# Autodesk Inventor assembly: MultiPassSCAN_outsideIn-DFMOD_SCAN_COLOR
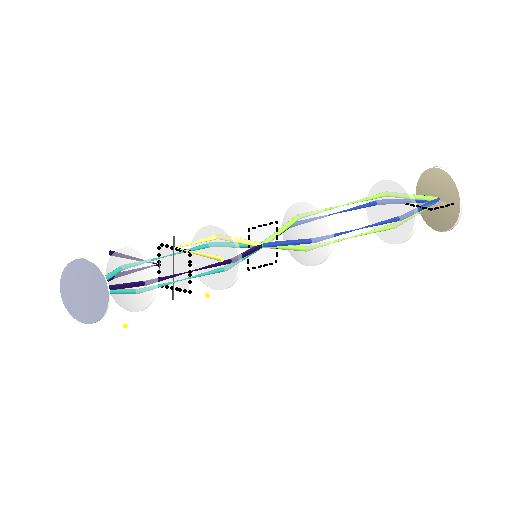
[picture p0: Inventor's stored thumbnail of the model, 512x512]
Saved by Autodesk Inventor 2026.1 (Build 301233000, 233)
## iProperties
Created: 2024-08-19
Part Number: MultiPassSCAN_outsideIn-DFMOD_SCAN_COLOR
Document SubType Name: Assembly
Designer: User
Author: User
## Documents named in this file (22)
- C:\Users\farin012\Downloads\fig4\fig4\MultiPassSCAN_outsideIn-DFMOD_SCAN_COLOR.iam
- C:\Users\farin012\Downloads\fig4\fig4\BB1-E02-Solidworks.ipt
- C:\Users\farin012\Downloads\fig4\fig4\LoopPlane1.ipt
- C:\Users\farin012\Downloads\fig4\fig4\LA1608-AB-Solidworks\LA1608-AB-2LOOP_grid.ipt
- C:\Users\farin012\Downloads\fig4\fig4\LOOP1_COLL.ipt
- C:\Users\farin012\Downloads\fig4\fig4\LOOP1_COLL_PREDEF1.ipt
- C:\Users\farin012\Downloads\fig4\fig4\LOOP1_COLL_POSTDEF1.ipt
- C:\Users\farin012\Downloads\fig4\fig4\deflection_plane.ipt
- C:\Users\farin012\Downloads\fig4\fig4\LOOP1_COLL_PREDEF2.ipt
- C:\Users\farin012\Downloads\fig4\fig4\LOOP1_COLL_POSTDEF2.ipt
- C:\Users\farin012\Downloads\fig4\fig4\LOOP2_COLL_PREDEF1.ipt
- C:\Users\farin012\Downloads\fig4\fig4\LOOP2_COLL_POSTDEF1.ipt
- C:\Users\farin012\Downloads\fig4\fig4\LOOP2_COLL_PREDEF2.ipt
- C:\Users\farin012\Downloads\fig4\fig4\LOOP2_COLL_POSTDEF2.ipt
- C:\Users\farin012\Downloads\fig4\fig4\LaserBeamEntry2_UNDEF.ipt
- C:\Users\farin012\Downloads\fig4\fig4\LaserBeamEntry2_LOOP1DEF1.ipt
- C:\Users\farin012\Downloads\fig4\fig4\LaserBeamEntry2_LOOP1DEF2.ipt
- C:\Users\farin012\Downloads\fig4\fig4\LaserBeamEntry2_LOOP2DEF1.ipt
- C:\Users\farin012\Downloads\fig4\fig4\LaserBeamEntry2_LOOP2DEF2.ipt
- C:\Users\farin012\Downloads\fig4\fig4\EntryMirror.ipt
- C:\Users\farin012\Downloads\fig4\fig4\ExitMirror.ipt
- C:\Users\farin012\Downloads\fig4\fig4\LaserBeamEntry2.ipt
## Components (46 placed, 21 different names)
1. BB1-E02-Solidworks:1 — Mate:115, Mate:125, Mate:126, Mate:127, Angle:6, Mate:128, Mate:147
2. BB1-E02-Solidworks:2 — Angle:5, Mate:137, Mate:138, Mate:232
3. LoopPlane1:1 — Mate:113
4. LA1608-AB-2LOOP_grid:1 — Flush:3, Mate:145, Mate:147, Mate:148, Mate:173, Mate:174, Mate:175, Mate:176, Mate:196, Flush:172, Mate:197, Flush:173, Mate:204, Flush:180, Mate:205, Flush:181
5. LA1608-AB-2LOOP_grid:2 — Flush:2, Mate:145, Mate:146, Mate:149, Mate:155, Mate:156, Mate:169, Mate:170, Mate:179, Mate:180, Mate:193, Mate:194, Mate:198, Flush:174, Mate:203, Flush:179, Mate:206, Flush:182, Mate:211, Flush:187
6. LA1608-AB-2LOOP_grid:3 — Flush:5, Mate:137, Mate:151, Mate:152, Mate:161, Mate:162, Mate:163, Mate:164, Mate:185, Mate:186, Mate:187, Mate:188, Mate:200, Flush:176, Mate:201, Flush:177, Mate:208, Flush:184, Mate:209, Flush:185
7. LA1608-AB-2LOOP_grid:4 — Flush:4, Mate:146, Mate:150, Mate:152, Mate:167, Mate:168, Mate:181, Mate:182, Mate:191, Mate:192, Mate:199, Flush:175, Mate:202, Flush:178, Mate:207, Flush:183, Mate:210, Flush:186
8. LOOP1_COLL:1 — Mate:125, Mate:126
9. LOOP1_COLL:2 — Mate:127, Mate:128
10. LOOP1_COLL_PREDEF1:1 — Mate:155, Mate:156
11. LOOP1_COLL_POSTDEF1:1
12. deflection_plane:1 — Mate:230, Flush:190, Flush:191
13. LOOP1_COLL_POSTDEF1:2 — Mate:161, Mate:162
14. LOOP1_COLL_POSTDEF1:3 — Mate:163, Mate:164
15. LOOP1_COLL_PREDEF2:1 — Mate:167, Mate:168
16. LOOP1_COLL_POSTDEF2:1 — Mate:169, Mate:170
17. LOOP2_COLL_PREDEF1:1 — Mate:173, Mate:174
18. LOOP2_COLL_PREDEF1:2 — Mate:175, Mate:176
19. LOOP2_COLL_PREDEF1:3 — Mate:179, Mate:180
20. LOOP2_COLL_POSTDEF1:1 — Mate:181, Mate:182
21. LOOP2_COLL_POSTDEF1:2 — Mate:185, Mate:186
22. LOOP2_COLL_PREDEF2:1 — Mate:187, Mate:188
23. LOOP2_COLL_PREDEF2:2 — Mate:191, Mate:192
24. LOOP2_COLL_POSTDEF2:1 — Mate:193, Mate:194
25. LaserBeamEntry2_UNDEF:1 — Mate:196, Flush:172, Mate:216, Mate:218, Mate:220, Mate:221
26. LaserBeamEntry2_UNDEF:2 — Mate:198, Flush:174
27. LaserBeamEntry2_UNDEF:3 — Mate:197, Flush:173
28. LaserBeamEntry2_LOOP1DEF1:1 — Mate:200, Flush:176
29. LaserBeamEntry2_LOOP1DEF1:2 — Mate:199, Flush:175
30. LaserBeamEntry2_LOOP1DEF1:3 — Mate:202, Flush:178, Flush:191
31. LaserBeamEntry2_LOOP1DEF1:4 — Mate:201, Flush:177
32. LaserBeamEntry2_LOOP1DEF2:1 — Mate:204, Flush:180
33. LaserBeamEntry2_LOOP1DEF2:2 — Mate:203, Flush:179
34. LaserBeamEntry2_LOOP1DEF2:3 — Mate:205, Flush:181
35. LaserBeamEntry2_LOOP1DEF2:4 — Mate:206, Flush:182
36. LaserBeamEntry2_LOOP2DEF1:1 — Mate:208, Flush:184
37. LaserBeamEntry2_LOOP2DEF1:2 — Mate:207, Flush:183
38. LaserBeamEntry2_LOOP2DEF1:3 — Mate:209, Flush:185
39. LaserBeamEntry2_LOOP2DEF1:4 — Mate:210, Flush:186
40. LaserBeamEntry2_LOOP2DEF2:1 — Mate:211, Flush:187, Mate:225
41. deflection_plane:2 — Mate:216, Mate:217, Mate:218, Mate:219, Mate:226
42. EntryMirror:1 — Mate:220, Angle:7, Mate:221, Mate:222, Flush:188
43. ExitMirror:1 — Mate:223, Mate:224, Mate:225, Flush:189
44. deflection_plane:3 — Mate:231, Angle:8, Mate:232
45. LaserBeamEntry2:1 — Mate:222, Flush:188
46. LaserBeamEntry2_LOOP2DEF2:2 — Mate:226, Flush:189
## Relationships (102: Mate 74, Flush 24, Angle 4)
- Mate:22
- Mate:23
- Mate:113: LoopPlane1:1
- Mate:115: BB1-E02-Solidworks:1
- Angle:5 (180 deg): BB1-E02-Solidworks:2
- Flush:2: LA1608-AB-2LOOP_grid:2
- Flush:3: LA1608-AB-2LOOP_grid:1
- Flush:4: LA1608-AB-2LOOP_grid:4
- Flush:5: LA1608-AB-2LOOP_grid:3
- Mate:125: BB1-E02-Solidworks:1 ↔ LOOP1_COLL:1
- Mate:126: BB1-E02-Solidworks:1 ↔ LOOP1_COLL:1
- Mate:127: BB1-E02-Solidworks:1 ↔ LOOP1_COLL:2
- Angle:6 (0 deg): BB1-E02-Solidworks:1
- Mate:128: BB1-E02-Solidworks:1 ↔ LOOP1_COLL:2
- Mate:137 (25 mm): BB1-E02-Solidworks:2 ↔ LA1608-AB-2LOOP_grid:3
- Mate:138: BB1-E02-Solidworks:2
- Mate:145 (-50 mm): LA1608-AB-2LOOP_grid:1 ↔ LA1608-AB-2LOOP_grid:2
- Mate:146 (50 mm): LA1608-AB-2LOOP_grid:2 ↔ LA1608-AB-2LOOP_grid:4
- Mate:147 (25 mm): BB1-E02-Solidworks:1 ↔ LA1608-AB-2LOOP_grid:1
- Mate:148: LA1608-AB-2LOOP_grid:1
- Mate:149: LA1608-AB-2LOOP_grid:2
- Mate:150: LA1608-AB-2LOOP_grid:4
- Mate:151: LA1608-AB-2LOOP_grid:3
- Mate:152 (-50 mm): LA1608-AB-2LOOP_grid:3 ↔ LA1608-AB-2LOOP_grid:4
- Mate:155: LA1608-AB-2LOOP_grid:2 ↔ LOOP1_COLL_PREDEF1:1
- Mate:156: LA1608-AB-2LOOP_grid:2 ↔ LOOP1_COLL_PREDEF1:1
- Mate:161: LA1608-AB-2LOOP_grid:3 ↔ LOOP1_COLL_POSTDEF1:2
- Mate:162: LA1608-AB-2LOOP_grid:3 ↔ LOOP1_COLL_POSTDEF1:2
- Mate:163: LA1608-AB-2LOOP_grid:3 ↔ LOOP1_COLL_POSTDEF1:3
- Mate:164: LA1608-AB-2LOOP_grid:3 ↔ LOOP1_COLL_POSTDEF1:3
- Mate:167: LA1608-AB-2LOOP_grid:4 ↔ LOOP1_COLL_PREDEF2:1
- Mate:168: LA1608-AB-2LOOP_grid:4 ↔ LOOP1_COLL_PREDEF2:1
- Mate:169: LA1608-AB-2LOOP_grid:2 ↔ LOOP1_COLL_POSTDEF2:1
- Mate:170: LA1608-AB-2LOOP_grid:2 ↔ LOOP1_COLL_POSTDEF2:1
- Mate:173: LA1608-AB-2LOOP_grid:1 ↔ LOOP2_COLL_PREDEF1:1
- Mate:174: LA1608-AB-2LOOP_grid:1 ↔ LOOP2_COLL_PREDEF1:1
- Mate:175: LA1608-AB-2LOOP_grid:1 ↔ LOOP2_COLL_PREDEF1:2
- Mate:176: LA1608-AB-2LOOP_grid:1 ↔ LOOP2_COLL_PREDEF1:2
- Mate:179: LA1608-AB-2LOOP_grid:2 ↔ LOOP2_COLL_PREDEF1:3
- Mate:180: LA1608-AB-2LOOP_grid:2 ↔ LOOP2_COLL_PREDEF1:3
- Mate:181: LA1608-AB-2LOOP_grid:4 ↔ LOOP2_COLL_POSTDEF1:1
- Mate:182: LA1608-AB-2LOOP_grid:4 ↔ LOOP2_COLL_POSTDEF1:1
- Mate:185: LA1608-AB-2LOOP_grid:3 ↔ LOOP2_COLL_POSTDEF1:2
- Mate:186: LA1608-AB-2LOOP_grid:3 ↔ LOOP2_COLL_POSTDEF1:2
- Mate:187: LA1608-AB-2LOOP_grid:3 ↔ LOOP2_COLL_PREDEF2:1
- Mate:188: LA1608-AB-2LOOP_grid:3 ↔ LOOP2_COLL_PREDEF2:1
- Mate:191: LA1608-AB-2LOOP_grid:4 ↔ LOOP2_COLL_PREDEF2:2
- Mate:192: LA1608-AB-2LOOP_grid:4 ↔ LOOP2_COLL_PREDEF2:2
- Mate:193: LA1608-AB-2LOOP_grid:2 ↔ LOOP2_COLL_POSTDEF2:1
- Mate:194: LA1608-AB-2LOOP_grid:2 ↔ LOOP2_COLL_POSTDEF2:1
- Mate:196: LA1608-AB-2LOOP_grid:1 ↔ LaserBeamEntry2_UNDEF:1
- Flush:172: LA1608-AB-2LOOP_grid:1 ↔ LaserBeamEntry2_UNDEF:1
- Mate:197: LA1608-AB-2LOOP_grid:1 ↔ LaserBeamEntry2_UNDEF:3
- Mate:198: LA1608-AB-2LOOP_grid:2 ↔ LaserBeamEntry2_UNDEF:2
- Flush:173: LA1608-AB-2LOOP_grid:1 ↔ LaserBeamEntry2_UNDEF:3
- Flush:174: LA1608-AB-2LOOP_grid:2 ↔ LaserBeamEntry2_UNDEF:2
- Mate:199: LA1608-AB-2LOOP_grid:4 ↔ LaserBeamEntry2_LOOP1DEF1:2
- Flush:175: LA1608-AB-2LOOP_grid:4 ↔ LaserBeamEntry2_LOOP1DEF1:2
- Mate:200: LA1608-AB-2LOOP_grid:3 ↔ LaserBeamEntry2_LOOP1DEF1:1
- Flush:176: LA1608-AB-2LOOP_grid:3 ↔ LaserBeamEntry2_LOOP1DEF1:1
- Mate:201: LA1608-AB-2LOOP_grid:3 ↔ LaserBeamEntry2_LOOP1DEF1:4
- Flush:177: LA1608-AB-2LOOP_grid:3 ↔ LaserBeamEntry2_LOOP1DEF1:4
- Mate:202: LA1608-AB-2LOOP_grid:4 ↔ LaserBeamEntry2_LOOP1DEF1:3
- Flush:178: LA1608-AB-2LOOP_grid:4 ↔ LaserBeamEntry2_LOOP1DEF1:3
- Mate:203: LA1608-AB-2LOOP_grid:2 ↔ LaserBeamEntry2_LOOP1DEF2:2
- Flush:179: LA1608-AB-2LOOP_grid:2 ↔ LaserBeamEntry2_LOOP1DEF2:2
- Mate:204: LA1608-AB-2LOOP_grid:1 ↔ LaserBeamEntry2_LOOP1DEF2:1
- Flush:180: LA1608-AB-2LOOP_grid:1 ↔ LaserBeamEntry2_LOOP1DEF2:1
- Mate:205: LA1608-AB-2LOOP_grid:1 ↔ LaserBeamEntry2_LOOP1DEF2:3
- Flush:181: LA1608-AB-2LOOP_grid:1 ↔ LaserBeamEntry2_LOOP1DEF2:3
- Mate:206: LA1608-AB-2LOOP_grid:2 ↔ LaserBeamEntry2_LOOP1DEF2:4
- Flush:182: LA1608-AB-2LOOP_grid:2 ↔ LaserBeamEntry2_LOOP1DEF2:4
- Mate:207: LA1608-AB-2LOOP_grid:4 ↔ LaserBeamEntry2_LOOP2DEF1:2
- Flush:183: LA1608-AB-2LOOP_grid:4 ↔ LaserBeamEntry2_LOOP2DEF1:2
- Mate:208: LA1608-AB-2LOOP_grid:3 ↔ LaserBeamEntry2_LOOP2DEF1:1
- Flush:184: LA1608-AB-2LOOP_grid:3 ↔ LaserBeamEntry2_LOOP2DEF1:1
- Mate:209: LA1608-AB-2LOOP_grid:3 ↔ LaserBeamEntry2_LOOP2DEF1:3
- Flush:185: LA1608-AB-2LOOP_grid:3 ↔ LaserBeamEntry2_LOOP2DEF1:3
- Mate:210: LA1608-AB-2LOOP_grid:4 ↔ LaserBeamEntry2_LOOP2DEF1:4
- Flush:186: LA1608-AB-2LOOP_grid:4 ↔ LaserBeamEntry2_LOOP2DEF1:4
- Mate:211: LA1608-AB-2LOOP_grid:2 ↔ LaserBeamEntry2_LOOP2DEF2:1
- Flush:187: LA1608-AB-2LOOP_grid:2 ↔ LaserBeamEntry2_LOOP2DEF2:1
- Mate:216: LaserBeamEntry2_UNDEF:1 ↔ deflection_plane:2
- Mate:217: deflection_plane:2
- Mate:218: LaserBeamEntry2_UNDEF:1 ↔ deflection_plane:2
- Mate:219: deflection_plane:2
- Mate:220: LaserBeamEntry2_UNDEF:1 ↔ EntryMirror:1
- Angle:7 (180 deg): EntryMirror:1
- Mate:221: LaserBeamEntry2_UNDEF:1 ↔ EntryMirror:1
- Mate:222: EntryMirror:1 ↔ LaserBeamEntry2:1
- Flush:188: EntryMirror:1 ↔ LaserBeamEntry2:1
- Mate:223: ExitMirror:1
- Mate:224: ExitMirror:1
- Mate:225: LaserBeamEntry2_LOOP2DEF2:1 ↔ ExitMirror:1
- Mate:226: deflection_plane:2 ↔ LaserBeamEntry2_LOOP2DEF2:2
- Flush:189: ExitMirror:1 ↔ LaserBeamEntry2_LOOP2DEF2:2
- Mate:230: deflection_plane:1
- Flush:190: deflection_plane:1
- Flush:191 (25 mm): deflection_plane:1 ↔ LaserBeamEntry2_LOOP1DEF1:3
- Mate:231: deflection_plane:3
- Angle:8 (90 deg): deflection_plane:3
- Mate:232 (5 mm): BB1-E02-Solidworks:2 ↔ deflection_plane:3
